# Autodesk Inventor assembly: HandLeft
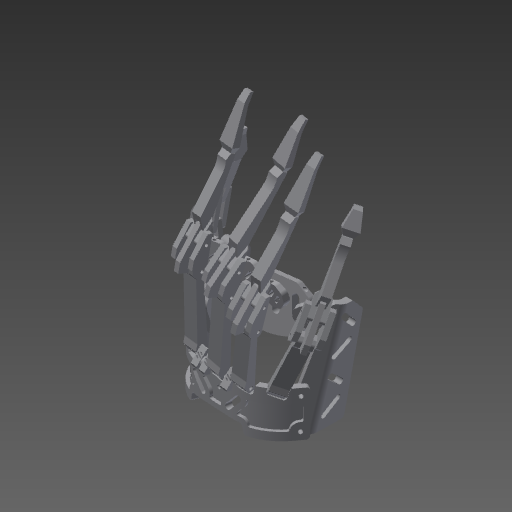
[picture p0: Inventor's stored thumbnail of the model, 512x512]
Saved by Autodesk Inventor 2020 (Build 240168000, 168)
## iProperties
Created: 2016-10-02
Part Number: HandLeft
Document SubType Name: Assembly
Designer: Val
Author: Val
## Documents named in this file (27)
- C:\Users\valer\Desktop\elysium-max-exoskeleton\src\Assemblies\HandRight.iam
- C:\Users\valer\Desktop\elysium-max-exoskeleton\src\DistPhalangeThumb.ipt
- C:\Users\valer\Desktop\elysium-max-exoskeleton\src\MetacarpusThumb.ipt
- C:\Users\valer\Desktop\elysium-max-exoskeleton\src\ProxPhalangeThumb.ipt
- C:\Users\valer\Desktop\elysium-max-exoskeleton\src\ThumbMount.ipt
- C:\Users\valer\Desktop\elysium-max-exoskeleton\src\DistPhalangeIndex.ipt
- C:\Users\valer\Desktop\elysium-max-exoskeleton\src\DistPhalangeMiddle.ipt
- C:\Users\valer\Desktop\elysium-max-exoskeleton\src\DistPhalangePinky.ipt
- C:\Users\valer\Desktop\elysium-max-exoskeleton\src\DistPhalangeRing.ipt
- C:\Users\valer\Desktop\elysium-max-exoskeleton\src\ProxPhalangeIndex.ipt
- C:\Users\valer\Desktop\elysium-max-exoskeleton\src\ProxPhalangeMiddle.ipt
- C:\Users\valer\Desktop\elysium-max-exoskeleton\src\ProxPhalangePinky.ipt
- C:\Users\valer\Desktop\elysium-max-exoskeleton\src\ProxPhalangeRing.ipt
- C:\Users\valer\Desktop\elysium-max-exoskeleton\src\MetacarpusIndex.ipt
- C:\Users\valer\Desktop\elysium-max-exoskeleton\src\MetacarpusMiddle.ipt
- C:\Users\valer\Desktop\elysium-max-exoskeleton\src\MetacarpusPinky.ipt
- C:\Users\valer\Desktop\elysium-max-exoskeleton\src\MetacarpusRing.ipt
- C:\Users\valer\Desktop\elysium-max-exoskeleton\src\Knuckle.ipt
- C:\Users\valer\Desktop\elysium-max-exoskeleton\src\KnuckleSide.ipt
- C:\Users\valer\Desktop\elysium-max-exoskeleton\src\IndexRouter.ipt
- C:\Users\valer\Desktop\elysium-max-exoskeleton\src\MiddleRouter.ipt
- C:\Users\valer\Desktop\elysium-max-exoskeleton\src\PinkyRouter.ipt
- C:\Users\valer\Desktop\elysium-max-exoskeleton\src\RingRouter.ipt
- C:\Users\valer\Desktop\elysium-max-exoskeleton\src\ThumbRouter.ipt
- C:\Users\valer\Desktop\elysium-max-exoskeleton\src\HandRibRight.ipt
- C:\Users\valer\Desktop\elysium-max-exoskeleton\src\HandShockPlateRight.ipt
- C:\Users\valer\Desktop\elysium-max-exoskeleton\src\ThumbShockPlateRight.ipt
## Components (39 placed, 26 different names)
1. DistPhalangeThumb:1 — Mate:9, Mate:10
2. MetacarpusThumb:1 — Mate:7, Mate:8, Mate:11, Mate:12, Mate:29, Mate:30, Mate:34, Mate:35
3. ProxPhalangeThumb:1 — Mate:9, Mate:10, Mate:13, Mate:14, Mate:31, Mate:36
4. ThumbMount:1 — Mate:7, Mate:8, Mate:78, Mate:79, Mate:80
5. DistPhalangeIndex:1 — Mate:23, Mate:46
6. DistPhalangeMiddle:1 — Mate:45, Mate:47
7. DistPhalangePinky:1 — Mate:66, Mate:67
8. DistPhalangeRing:1 — Mate:53, Mate:54
9. ProxPhalangeIndex:1 — Mate:18, Mate:19, Mate:22, Mate:23, Mate:27, Mate:46
10. ProxPhalangeMiddle:1 — Mate:37, Mate:38, Mate:41, Mate:44, Mate:45, Mate:47
11. ProxPhalangePinky:1 — Mate:64, Mate:65, Mate:66, Mate:67, Mate:70, Mate:73
12. ProxPhalangeRing:1 — Mate:51, Mate:52, Mate:53, Mate:54, Mate:57, Mate:60
13. MetacarpusIndex:1 — Mate:16, Mate:17, Mate:20, Mate:21, Mate:25, Mate:26, Mate:81, Angle:1
14. MetacarpusMiddle:1 — Mate:32, Mate:33, Mate:39, Mate:40, Mate:42, Mate:43, Mate:82, Angle:2
15. MetacarpusPinky:1 — Mate:62, Mate:63, Mate:68, Mate:69, Mate:71, Mate:72, Mate:84, Angle:4
16. MetacarpusRing:1 — Mate:49, Mate:50, Mate:55, Mate:56, Mate:58, Mate:59, Mate:83, Angle:3
17. Knuckle:1 — Mate:11, Mate:12, Mate:13, Mate:14
18. Knuckle:2 — Mate:16, Mate:17, Mate:18, Mate:19
19. Knuckle:3 — Mate:32, Mate:33, Mate:37, Mate:38
20. Knuckle:4 — Mate:49, Mate:50, Mate:51, Mate:52
21. Knuckle:5 — Mate:62, Mate:63, Mate:64, Mate:65
22. KnuckleSide:1 — Mate:42, Mate:43, Mate:44
23. KnuckleSide:2 — Mate:39, Mate:40, Mate:41
24. KnuckleSide:3 — Mate:55, Mate:56, Mate:57
25. KnuckleSide:4 — Mate:58, Mate:59, Mate:60
26. KnuckleSide:5 — Mate:29, Mate:30, Mate:31
27. KnuckleSide:6 — Mate:34, Mate:35, Mate:36
28. KnuckleSide:7 — Mate:68, Mate:69, Mate:70
29. KnuckleSide:8 — Mate:71, Mate:72, Mate:73
30. KnuckleSide:9 — Mate:25, Mate:26, Mate:27
31. KnuckleSide:10 — Mate:20, Mate:21, Mate:22
32. IndexRouter:1
33. MiddleRouter:1
34. PinkyRouter:1
35. RingRouter:1
36. ThumbRouter:1
37. HandRibRight:1 — Mate:76, Mate:77
38. HandShockPlateRight:1 — Mate:74, Mate:75, Mate:76, Mate:77, Mate:81, Angle:1, Mate:82, Angle:2, Mate:83, Angle:3, Mate:84, Angle:4
39. ThumbShockPlateRight:1 — Mate:74, Mate:75, Mate:78, Mate:79, Mate:80
## Relationships (77: Mate 73, Angle 4)
- Mate:7: MetacarpusThumb:1 ↔ ThumbMount:1
- Mate:8: MetacarpusThumb:1 ↔ ThumbMount:1
- Mate:9: DistPhalangeThumb:1 ↔ ProxPhalangeThumb:1
- Mate:10: DistPhalangeThumb:1 ↔ ProxPhalangeThumb:1
- Mate:11: MetacarpusThumb:1 ↔ Knuckle:1
- Mate:12: MetacarpusThumb:1 ↔ Knuckle:1
- Mate:13: ProxPhalangeThumb:1 ↔ Knuckle:1
- Mate:14: ProxPhalangeThumb:1 ↔ Knuckle:1
- Mate:16: MetacarpusIndex:1 ↔ Knuckle:2
- Mate:17: MetacarpusIndex:1 ↔ Knuckle:2
- Mate:18: ProxPhalangeIndex:1 ↔ Knuckle:2
- Mate:19: ProxPhalangeIndex:1 ↔ Knuckle:2
- Mate:20: MetacarpusIndex:1 ↔ KnuckleSide:10
- Mate:21: MetacarpusIndex:1 ↔ KnuckleSide:10
- Mate:22: ProxPhalangeIndex:1 ↔ KnuckleSide:10
- Mate:23: DistPhalangeIndex:1 ↔ ProxPhalangeIndex:1
- Mate:25: MetacarpusIndex:1 ↔ KnuckleSide:9
- Mate:26: MetacarpusIndex:1 ↔ KnuckleSide:9
- Mate:27: ProxPhalangeIndex:1 ↔ KnuckleSide:9
- Mate:29: MetacarpusThumb:1 ↔ KnuckleSide:5
- Mate:30: MetacarpusThumb:1 ↔ KnuckleSide:5
- Mate:31: ProxPhalangeThumb:1 ↔ KnuckleSide:5
- Mate:32: MetacarpusMiddle:1 ↔ Knuckle:3
- Mate:33: MetacarpusMiddle:1 ↔ Knuckle:3
- Mate:34: MetacarpusThumb:1 ↔ KnuckleSide:6
- Mate:35: MetacarpusThumb:1 ↔ KnuckleSide:6
- Mate:36: ProxPhalangeThumb:1 ↔ KnuckleSide:6
- Mate:37: ProxPhalangeMiddle:1 ↔ Knuckle:3
- Mate:38: ProxPhalangeMiddle:1 ↔ Knuckle:3
- Mate:39: MetacarpusMiddle:1 ↔ KnuckleSide:2
- Mate:40: MetacarpusMiddle:1 ↔ KnuckleSide:2
- Mate:41: ProxPhalangeMiddle:1 ↔ KnuckleSide:2
- Mate:42: MetacarpusMiddle:1 ↔ KnuckleSide:1
- Mate:43: MetacarpusMiddle:1 ↔ KnuckleSide:1
- Mate:44: ProxPhalangeMiddle:1 ↔ KnuckleSide:1
- Mate:45: DistPhalangeMiddle:1 ↔ ProxPhalangeMiddle:1
- Mate:46: DistPhalangeIndex:1 ↔ ProxPhalangeIndex:1
- Mate:47: DistPhalangeMiddle:1 ↔ ProxPhalangeMiddle:1
- Mate:49: MetacarpusRing:1 ↔ Knuckle:4
- Mate:50: MetacarpusRing:1 ↔ Knuckle:4
- Mate:51: ProxPhalangeRing:1 ↔ Knuckle:4
- Mate:52: ProxPhalangeRing:1 ↔ Knuckle:4
- Mate:53: DistPhalangeRing:1 ↔ ProxPhalangeRing:1
- Mate:54: DistPhalangeRing:1 ↔ ProxPhalangeRing:1
- Mate:55: MetacarpusRing:1 ↔ KnuckleSide:3
- Mate:56: MetacarpusRing:1 ↔ KnuckleSide:3
- Mate:57: ProxPhalangeRing:1 ↔ KnuckleSide:3
- Mate:58: MetacarpusRing:1 ↔ KnuckleSide:4
- Mate:59: MetacarpusRing:1 ↔ KnuckleSide:4
- Mate:60: ProxPhalangeRing:1 ↔ KnuckleSide:4
- Mate:62: MetacarpusPinky:1 ↔ Knuckle:5
- Mate:63: MetacarpusPinky:1 ↔ Knuckle:5
- Mate:64: ProxPhalangePinky:1 ↔ Knuckle:5
- Mate:65: ProxPhalangePinky:1 ↔ Knuckle:5
- Mate:66: DistPhalangePinky:1 ↔ ProxPhalangePinky:1
- Mate:67: DistPhalangePinky:1 ↔ ProxPhalangePinky:1
- Mate:68: MetacarpusPinky:1 ↔ KnuckleSide:7
- Mate:69: MetacarpusPinky:1 ↔ KnuckleSide:7
- Mate:70: ProxPhalangePinky:1 ↔ KnuckleSide:7
- Mate:71: MetacarpusPinky:1 ↔ KnuckleSide:8
- Mate:72: MetacarpusPinky:1 ↔ KnuckleSide:8
- Mate:73: ProxPhalangePinky:1 ↔ KnuckleSide:8
- Mate:74: HandShockPlateRight:1 ↔ ThumbShockPlateRight:1
- Mate:75: HandShockPlateRight:1 ↔ ThumbShockPlateRight:1
- Mate:76: HandRibRight:1 ↔ HandShockPlateRight:1
- Mate:77: HandRibRight:1 ↔ HandShockPlateRight:1
- Mate:78: ThumbMount:1 ↔ ThumbShockPlateRight:1
- Mate:79: ThumbMount:1 ↔ ThumbShockPlateRight:1
- Mate:80: ThumbMount:1 ↔ ThumbShockPlateRight:1
- Mate:81: MetacarpusIndex:1 ↔ HandShockPlateRight:1
- Angle:1 (0 deg): MetacarpusIndex:1 ↔ HandShockPlateRight:1
- Mate:82: MetacarpusMiddle:1 ↔ HandShockPlateRight:1
- Angle:2 (0 deg): MetacarpusMiddle:1 ↔ HandShockPlateRight:1
- Mate:83: MetacarpusRing:1 ↔ HandShockPlateRight:1
- Angle:3 (0 deg): MetacarpusRing:1 ↔ HandShockPlateRight:1
- Mate:84: MetacarpusPinky:1 ↔ HandShockPlateRight:1
- Angle:4 (0 deg): MetacarpusPinky:1 ↔ HandShockPlateRight:1
